# Autodesk Inventor assembly: Head
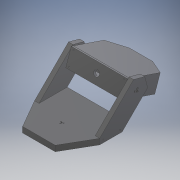
[picture p0: Inventor's stored thumbnail of the model, 180x180]
Saved by Autodesk Inventor 2017 (Build 210142000, 142)
## iProperties
Created: 2018-10-18
Part Number: Head
Document SubType Name: Assembly
Designer: Dell
Author: Dell
## Documents named in this file (9)
- C:\Users\Dell\Documents\GitHub\tr2\Head\Head.iam
- C:\Users\Dell\Documents\GitHub\tr2\Head\HA01.ipt
- C:\Users\Dell\Documents\GitHub\tr2\Head\Orbbec Astra\Orbbec Astra.iam
- C:\Users\Dell\Documents\GitHub\tr2\Head\HA02.ipt
- C:\Users\Dell\Documents\GitHub\tr2\Wheel Assembly\6mm Mounting Hub, thin.ipt
- C:\Users\Dell\Documents\GitHub\tr2\Head\HA03.ipt
- C:\Users\Dell\Documents\GitHub\tr2\Base\37d-gearmotor-50-70-encoder.ipt
- C:\Users\Dell\Documents\GitHub\tr2\Head\HA04.ipt
- C:\Users\Dell\Documents\GitHub\tr2\Head\HA05.ipt
## Components (9 placed, 8 different names)
1. HA01:1 — Mate:1, Flush:1, Mate:11, Mate:12, Mate:13, Mate:14, Mate:16, Mate:17, Mate:28, Mate:29
2. HA02:1 — Mate:4, Mate:8, Mate:9, Mate:10, Mate:21, Mate:22, Mate:23, Mate:24, Mate:25, Mate:26
3. HA03:1 — Mate:11, Mate:12, Mate:13
4. Orbbec Astra:1 [sub-assembly] — Mate:1, Flush:1
5. 6mm Mounting Hub, thin:1 — Mate:8, Mate:9, Mate:10
6. 37d-gearmotor-50-70-encoder:1 — Mate:14, Mate:16, Mate:17, Mate:19
7. 6mm Mounting Hub, thin:2 — Mate:19, Mate:27
8. HA04:1 — Mate:21, Mate:22, Mate:23, Mate:28
9. HA05:1 — Mate:24, Mate:25, Mate:26, Mate:27, Mate:29
## Relationships (22: Mate 21, Flush 1)
- Mate:1 (2 mm): HA01:1 ↔ Orbbec Astra:1
- Flush:1 (-20 mm): HA01:1 ↔ Orbbec Astra:1
- Mate:4: HA02:1
- Mate:8: HA02:1 ↔ 6mm Mounting Hub, thin:1
- Mate:9: HA02:1 ↔ 6mm Mounting Hub, thin:1
- Mate:10: HA02:1 ↔ 6mm Mounting Hub, thin:1
- Mate:11: HA01:1 ↔ HA03:1
- Mate:12: HA01:1 ↔ HA03:1
- Mate:13: HA01:1 ↔ HA03:1
- Mate:14: HA01:1 ↔ 37d-gearmotor-50-70-encoder:1
- Mate:16: HA01:1 ↔ 37d-gearmotor-50-70-encoder:1
- Mate:17: HA01:1 ↔ 37d-gearmotor-50-70-encoder:1
- Mate:19: 37d-gearmotor-50-70-encoder:1 ↔ 6mm Mounting Hub, thin:2
- Mate:21: HA02:1 ↔ HA04:1
- Mate:22: HA02:1 ↔ HA04:1
- Mate:23: HA02:1 ↔ HA04:1
- Mate:24: HA02:1 ↔ HA05:1
- Mate:25: HA02:1 ↔ HA05:1
- Mate:26: HA02:1 ↔ HA05:1
- Mate:27: 6mm Mounting Hub, thin:2 ↔ HA05:1
- Mate:28: HA01:1 ↔ HA04:1
- Mate:29: HA01:1 ↔ HA05:1
